# Autodesk Inventor assembly: wheel7
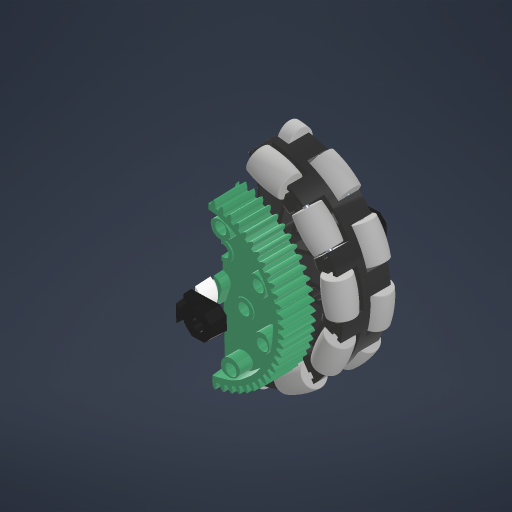
[picture p0: Inventor's stored thumbnail of the model, 512x512]
Saved by Autodesk Inventor 2024 (Build 280153000, 153)
## iProperties
Created: 2023-08-12
Part Number: wheel7
Document SubType Name: Assembly
Designer: macbook
Author: macbook
## Documents named in this file (15)
- \\Mac\Home\Desktop\code\7899V-VRC-OVER-UNDER\Cad\VEX-CAD-Inventor-1.4.0\Assembly\v0.2\wheel7.iam
- \\Mac\Home\Desktop\code\7899V-VRC-OVER-UNDER\Cad\VEX-CAD-Inventor-1.4.0\Motion\Wheels\Omni Wheel\3.25 Omni AS, Circle.iam
- \\Mac\Home\Desktop\code\7899V-VRC-OVER-UNDER\Cad\VEX-CAD-Inventor-1.4.0\Motion\Wheels\Omni Wheel.iam
- \\Mac\Home\Desktop\code\7899V-VRC-OVER-UNDER\Cad\VEX-CAD-Inventor-1.4.0\Motion\Shaft LS\Bearing Flat.ipt
- \\Mac\Home\Desktop\code\7899V-VRC-OVER-UNDER\Cad\VEX-CAD-Inventor-1.4.0\Structure\Hardware\Screw Steel - Star\SScrew Star Smooth .500.ipt
- \\Mac\Home\Desktop\code\7899V-VRC-OVER-UNDER\Cad\VEX-CAD-Inventor-1.4.0\Structure\Hardware\Screw Steel - Star.ipt
- \\Mac\Home\Desktop\code\7899V-VRC-OVER-UNDER\Cad\VEX-CAD-Inventor-1.4.0\Motion\Spacers\Spacer Nylon .313 OD\NSpacer .313 OD x .250.ipt
- \\Mac\Home\Desktop\code\7899V-VRC-OVER-UNDER\Cad\VEX-CAD-Inventor-1.4.0\Motion\Spacers\Spacer Nylon .313 OD.ipt
- \\Mac\Home\Desktop\code\7899V-VRC-OVER-UNDER\Cad\VEX-CAD-Inventor-1.4.0\Motion\Spacers\Spacer Nylon .500 OD\NSpacer White .500 OD x .250.ipt
- \\Mac\Home\Desktop\code\7899V-VRC-OVER-UNDER\Cad\VEX-CAD-Inventor-1.4.0\Motion\Spacers\Spacer Nylon .500 OD.ipt
- \\Mac\Home\Desktop\code\7899V-VRC-OVER-UNDER\Cad\VEX-CAD-Inventor-1.4.0\Motion\Spacers\Washer Teflon\TWasher .375 OD x .03125.ipt
- \\Mac\Home\Desktop\code\7899V-VRC-OVER-UNDER\Cad\VEX-CAD-Inventor-1.4.0\Motion\Spacers\Washer Teflon.ipt
- \\Mac\Home\Desktop\code\7899V-VRC-OVER-UNDER\Cad\VEX-CAD-Inventor-1.4.0\Structure\Hardware\Screw Steel - Star\SScrew Star Smooth 2.250.ipt
- \\Mac\Home\Desktop\code\7899V-VRC-OVER-UNDER\Cad\VEX-CAD-Inventor-1.4.0\Motion\Gears\HS Gear\HS 60T Gear, Circle Insert.iam
- \\Mac\Home\Desktop\code\7899V-VRC-OVER-UNDER\Cad\VEX-CAD-Inventor-1.4.0\Motion\Spacers\Spacer Nylon .313 OD\NSpacer .313 OD x .500.ipt
## Components (12 placed, 9 different names)
1. 3.25 Omni AS, Circle:1 [sub-assembly] — Insert:18
2. Bearing Flat:1
3. Bearing Flat:2
4. SScrew Star Smooth .500:1
5. NSpacer .313 OD x .250:1 — Insert:7
6. HS 60T Gear, Circle Insert:1 [sub-assembly] — Insert:7, Insert:17
7. NSpacer White .500 OD x .250:1 — Insert:17
8. SScrew Star Smooth 2.250:4
9. NSpacer .313 OD x .500:2 — Insert:18, Insert:21
10. TWasher .375 OD x .03125:1 — Insert:19
11. TWasher .375 OD x .03125:2 — Insert:19, Insert:20
12. TWasher .375 OD x .03125:3 — Insert:20, Insert:21
## Relationships (12: Insert 12)
- [Insert] (1.5875 mm): Bearing Flat:1 ↔ NSpacer White .500 OD x .250:1
- [Insert] (1.5875 mm): Bearing Flat:2 ↔ SScrew Star Smooth .500:1
- [Insert] (57.15 mm): Bearing Flat:1 ↔ Bearing Flat:2
- [Insert] (57.15 mm): Bearing Flat:1 ↔ Bearing Flat:2
- [Insert]: 3.25 Omni AS, Circle:1 ↔ NSpacer .313 OD x .250:1
- Insert:7: NSpacer .313 OD x .250:1 ↔ HS 60T Gear, Circle Insert:1
- [Insert]: Bearing Flat:1 ↔ SScrew Star Smooth 2.250:4
- Insert:17: HS 60T Gear, Circle Insert:1 ↔ NSpacer White .500 OD x .250:1
- Insert:18: 3.25 Omni AS, Circle:1 ↔ NSpacer .313 OD x .500:2
- Insert:19: TWasher .375 OD x .03125:1 ↔ TWasher .375 OD x .03125:2
- Insert:20: TWasher .375 OD x .03125:2 ↔ TWasher .375 OD x .03125:3
- Insert:21: NSpacer .313 OD x .500:2 ↔ TWasher .375 OD x .03125:3
